# Autodesk Inventor assembly: ASY DS-B beam 2
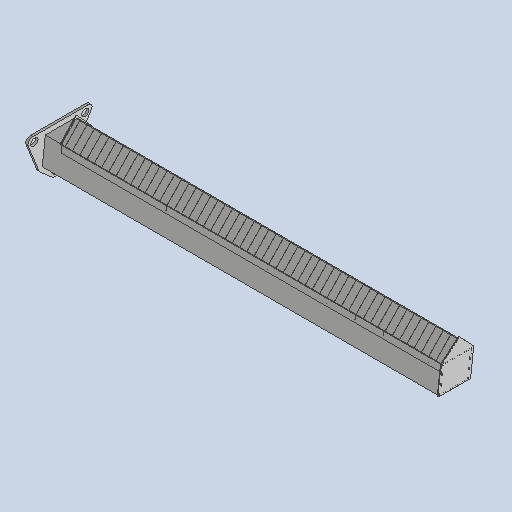
[picture p0: Inventor's stored thumbnail of the model, 512x512]
Saved by Autodesk Inventor 2025 (Build 290162010, 162A)
## iProperties
Created: 2025-02-18
Part Number: ASY DS-B beam 2
Document SubType Name: Assembly
Designer: admin
Author: admin
## Documents named in this file (6)
- C:\Users\DELL\YandexDisk-badmisterfox\home pc\Inventor\filter-distribution-system\ASY DS-B beam 2.iam
- C:\Users\DELL\YandexDisk-badmisterfox\home pc\Inventor\filter-distribution-system\DS-B-1101 beam 2.ipt
- C:\Users\DELL\YandexDisk-badmisterfox\home pc\Inventor\filter-distribution-system\DS-B-1102 roof 2.ipt
- C:\Users\DELL\YandexDisk-badmisterfox\home pc\Inventor\filter-distribution-system\DS-B-501 beam flange.ipt
- C:\Users\DELL\YandexDisk-badmisterfox\home pc\Inventor\filter-distribution-system\DS-B-502 CAPhouse.ipt
- C:\Users\DELL\YandexDisk-badmisterfox\home pc\Inventor\filter-distribution-system\DS-B-503 CAP.ipt
## Components (5 placed, 5 different names)
1. DS-B-1101 beam 2:1 — Flush:4, Flush:3, Mate:2, Flush:6, Mate:1, Flush:1, Mate:6, Rigid:1, Rigid:2
2. DS-B-1102 roof 2:1 — Flush:6, Mate:1, Flush:1, Mate:7
3. Part1:1 — Rigid:1
4. MNT-CDF-604 CAP:1 — Mate:3, Rigid:2
5. MNT-CDF-605 CAP:1 — Mate:7, Mate:6, Mate:5
## Relationships (12: Mate 6, Flush 4, WeldJoint 2)
- Flush:4: DS-B-1101 beam 2:1
- Flush:3: DS-B-1101 beam 2:1
- Mate:2: DS-B-1101 beam 2:1
- Flush:6: DS-B-1101 beam 2:1 ↔ DS-B-1102 roof 2:1
- Mate:1: DS-B-1101 beam 2:1 ↔ DS-B-1102 roof 2:1
- Flush:1: DS-B-1101 beam 2:1 ↔ DS-B-1102 roof 2:1
- Mate:3: MNT-CDF-604 CAP:1
- Mate:7: DS-B-1102 roof 2:1 ↔ MNT-CDF-605 CAP:1
- Mate:6: DS-B-1101 beam 2:1 ↔ MNT-CDF-605 CAP:1
- Mate:5: MNT-CDF-605 CAP:1
- Rigid:1 [WeldJoint]: DS-B-1101 beam 2:1 ↔ Part1:1
- Rigid:2 [WeldJoint]: DS-B-1101 beam 2:1 ↔ MNT-CDF-604 CAP:1
